# Autodesk Inventor assembly: plotter_new
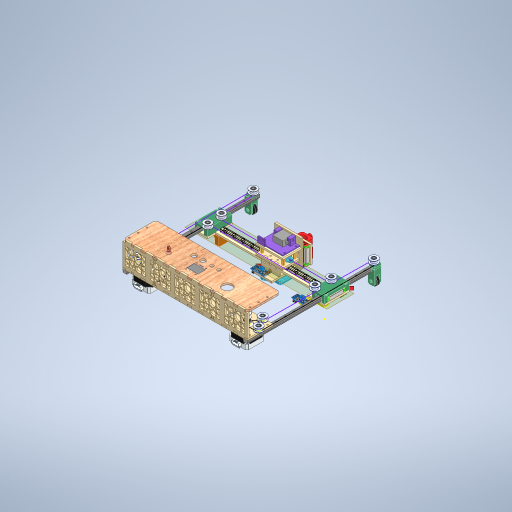
[picture p0: Inventor's stored thumbnail of the model, 512x512]
Saved by Autodesk Inventor 2024 (Build 280153000, 153)
## iProperties
Created: 2025-12-22
Part Number: plotter_new
Document SubType Name: Assembly
Designer: DELL
Author: DELL
## Documents named in this file (40)
- C:\Users\ejenie\reposGits\VSOSH25-26\models\plotter\plotter_actual\plotter_new.iam
- C:\Users\ejenie\reposGits\VSOSH25-26\models\plotter\plotter_actual\MGN9-H.ipt
- C:\Users\ejenie\reposGits\VSOSH25-26\models\plotter\plotter_actual\рельса.ipt
- C:\Users\ejenie\reposGits\VSOSH25-26\models\plotter\plotter_actual\Stepper motor Nema 17 (17HS2408).ipt
- C:\Users\ejenie\reposGits\VSOSH25-26\models\plotter\plotter_actual\центр_рейка.ipt
- C:\Users\ejenie\reposGits\VSOSH25-26\models\plotter\plotter_actual\креп_мотора.ipt
- C:\Users\ejenie\reposGits\VSOSH25-26\models\plotter\plotter_actual\Ролик с резьбой GT2 на моторы.ipt
- C:\Users\ejenie\reposGits\VSOSH25-26\models\plotter\plotter_actual\Сборка ролик с подшипником.ipt
- C:\Users\ejenie\reposGits\VSOSH25-26\models\plotter\plotter_actual\ограничитель.ipt
- C:\Users\ejenie\reposGits\VSOSH25-26\models\plotter\plotter_actual\рельса_центр.ipt
- C:\Users\ejenie\reposGits\VSOSH25-26\models\plotter\plotter_actual\Ролик с резьбой GT2 на моторы_MIR1.ipt
- C:\Users\ejenie\reposGits\VSOSH25-26\models\plotter\plotter_actual\Сборка ролик с подшипником_MIR3.ipt
- C:\Users\ejenie\reposGits\VSOSH25-26\models\plotter\plotter_actual\ограничитель_MIR.ipt
- C:\Users\ejenie\reposGits\VSOSH25-26\models\plotter\plotter_actual\креп_центр_м2.ipt
- C:\Users\ejenie\reposGits\VSOSH25-26\models\plotter\plotter_actual\Сборка ролик с подшипником_MIR4.ipt
- C:\Users\ejenie\reposGits\VSOSH25-26\models\plotter\plotter_actual\колесо.ipt
- C:\Users\ejenie\reposGits\VSOSH25-26\models\plotter\plotter_actual\концевик.ipt
- C:\Users\ejenie\reposGits\VSOSH25-26\models\plotter\plotter_actual\TCRT5000.ipt
- C:\Users\ejenie\reposGits\VSOSH25-26\models\plotter\plotter_actual\креп_опт.ipt
- C:\Users\ejenie\reposGits\VSOSH25-26\models\plotter\plotter_actual\креп_концевика.ipt
- C:\Users\ejenie\reposGits\VSOSH25-26\models\plotter\plotter_actual\креп_центр_м2_MIR1.ipt
- C:\Users\ejenie\reposGits\VSOSH25-26\models\plotter\plotter_actual\ремень.ipt
- C:\Users\ejenie\reposGits\VSOSH25-26\models\plotter\пол_каретки.ipt
- C:\Users\ejenie\reposGits\VSOSH25-26\models\plotter\стена_каретки.ipt
- C:\Users\ejenie\reposGits\VSOSH25-26\models\plotter\дно_каретки.ipt
- C:\Users\ejenie\reposGits\VSOSH25-26\models\plotter\plotter_actual\крепление_ремня_новое.ipt
- C:\Users\ejenie\reposGits\VSOSH25-26\models\plotter\plotter_actual\стойка.ipt
- C:\Users\ejenie\reposGits\VSOSH25-26\models\plotter\plotter_actual\креп_сервы.ipt
- C:\Users\ejenie\reposGits\VSOSH25-26\models\plotter\plotter_actual\JX Servo PDI-HV2006MG.ipt
- C:\Users\ejenie\reposGits\VSOSH25-26\models\plotter\plotter_actual\стена_для_рельс.ipt
- C:\Users\ejenie\reposGits\VSOSH25-26\models\plotter\plotter_actual\рельса_мини.ipt
- C:\Users\ejenie\reposGits\VSOSH25-26\models\plotter\plotter_actual\стена_движения_каретки_з.ipt
- C:\Users\ejenie\reposGits\VSOSH25-26\models\plotter\plotter_actual\креп_мотора (1).ipt
- C:\Users\ejenie\reposGits\VSOSH25-26\models\plotter\plotter_actual\креп_маркера.ipt
- C:\Users\ejenie\reposGits\VSOSH25-26\models\plotter\plotter_actual\каретки_потолок.ipt
- C:\Users\ejenie\reposGits\VSOSH25-26\models\plotter\plotter_actual\ширма.ipt
- C:\Users\ejenie\reposGits\VSOSH25-26\models\plotter\plotter_actual\line_sens_fixator.ipt
- C:\Users\ejenie\reposGits\VSOSH25-26\models\plotter\plotter_actual\I2C OLED 128Ч64 Display Module.ipt
- C:\Users\ejenie\reposGits\VSOSH25-26\models\plotter\plotter_actual\RCL371-1-1-12.ipt
- C:\Users\ejenie\reposGits\VSOSH25-26\models\plotter\plotter_actual\upor_koncevik.ipt
## Components (61 placed, 39 different names)
1. рельса:1 — Совмещение:1, Совмещение:11, Заподлицо:7, Совмещение:12, Заподлицо:9, Совмещение:62, Совмещение:63, Совмещение:90, Совмещение:91, Заподлицо:25, Совмещение:106
2. Stepper motor Nema 17 (17HS2408):2 — Заподлицо:7, Совмещение:12, Заподлицо:18, Совмещение:18, Заподлицо:25
3. рельса:2 — Заподлицо:13, Заподлицо:15, Совмещение:15, Совмещение:16, Заподлицо:16, Совмещение:50, Совмещение:51, Заподлицо:26, Совмещение:107
4. MGN9-H:2 — Совмещение:49
5. Stepper motor Nema 17 (17HS2408):3 — Заподлицо:15, Совмещение:15, Совмещение:60, Заподлицо:26, Совмещение:199
6. креп_мотора:1 — Заподлицо:18, Совмещение:19, Совмещение:96, Совмещение:97, Совмещение:98, Совмещение:99, Совмещение:244, Заподлицо:45, Заподлицо:46, Совмещение:299, Совмещение:300, Совмещение:301, Совмещение:302, Совмещение:303, Совмещение:304, Совмещение:305
7. Ролик с резьбой GT2 на моторы:1 — Совмещение:18, Совмещение:19
8. Сборка ролик с подшипником:1 — Совмещение:299, Совмещение:300
9. ограничитель:1 — Совмещение:90, Совмещение:91, Совмещение:92, Совмещение:93, Совмещение:102, Совмещение:103, Совмещение:106
10. Сборка ролик с подшипником:2 — Совмещение:92, Совмещение:93
11. Сборка ролик с подшипником:4 — Совмещение:160, Совмещение:161
12. Сборка ролик с подшипником:5 — Совмещение:162, Совмещение:166
13. рельса_центр:1 — Совмещение:37, Совмещение:38, Совмещение:52, Заподлицо:23, Совмещение:154
14. MGN9-H:3 — Совмещение:37, Совмещение:38, Совмещение:245, Совмещение:246, Совмещение:247
15. Ролик с резьбой GT2 на моторы_MIR1:1 — Совмещение:60, Совмещение:199
16. ограничитель_MIR:1 — Совмещение:39, Совмещение:40, Совмещение:50, Совмещение:51, Совмещение:104, Совмещение:105, Совмещение:107
17. Сборка ролик с подшипником_MIR3:2 — Совмещение:39, Совмещение:40
18. центр_рейка:1 — Совмещение:49, Совмещение:52, Заподлицо:23, Совмещение:66, Совмещение:67, Совмещение:127, Совмещение:136, Совмещение:146, Совмещение:147, Совмещение:149, Совмещение:155, Совмещение:156, Совмещение:157, Совмещение:158, Совмещение:200, Совмещение:201, Совмещение:202, Совмещение:322, Совмещение:323
19. MGN9-H:4 — Совмещение:62, Совмещение:63, Совмещение:66, Совмещение:67, Совмещение:127
20. Сборка ролик с подшипником_MIR4:1 — Совмещение:150, Совмещение:153
21. Сборка ролик с подшипником_MIR4:2 — Совмещение:152, Совмещение:165
22. Сборка ролик с подшипником:6 — Совмещение:96, Совмещение:97
23. Сборка ролик с подшипником:7 — Совмещение:98, Совмещение:99
24. Сборка ролик с подшипником:8 — Совмещение:301, Совмещение:302
25. колесо:1 — Совмещение:102, Совмещение:103
26. колесо:2 — Совмещение:104, Совмещение:105
27. концевик:1 — Совмещение:133, Совмещение:134, Совмещение:135
28. креп_центр_м2:1 — Совмещение:147, Совмещение:149, Совмещение:150, Совмещение:152, Совмещение:153, Совмещение:154, Совмещение:165
29. креп_концевика:2 — Совмещение:133, Совмещение:134, Совмещение:135, Совмещение:136, Совмещение:146, Совмещение:155
30. креп_центр_м2_MIR1:1 — Совмещение:156, Совмещение:157, Совмещение:158, Совмещение:160, Совмещение:161, Совмещение:162, Совмещение:166, Заподлицо:27
31. ремень:1 — Заподлицо:27
32. TCRT5000:3 — Совмещение:203, Заподлицо:31, Совмещение:204
33. креп_опт:1 — Совмещение:200, Совмещение:201, Совмещение:202, Совмещение:203, Заподлицо:31, Совмещение:204
34. креп_мотора (1):1 — Совмещение:244, Заподлицо:45, Заподлицо:46, Заподлицо:54, Совмещение:319, Совмещение:320, Совмещение:321
35. дно_каретки:1 — Совмещение:262, Совмещение:263, Заподлицо:50, Совмещение:264, Совмещение:265, Совмещение:270, Совмещение:271, Совмещение:272, Совмещение:310, Совмещение:311, Совмещение:312
36. пол_каретки:1 — Совмещение:245, Совмещение:246, Совмещение:247, Совмещение:248, Совмещение:250, Заподлицо:48, Совмещение:251, Заподлицо:49, Совмещение:252, Совмещение:253, Совмещение:254, Совмещение:255, Совмещение:256, Совмещение:257, Совмещение:258, Совмещение:259, Совмещение:260, Совмещение:268, Совмещение:269
37. стена_каретки:1 — Совмещение:248, Заподлицо:49, Совмещение:252
38. стена_каретки:2 — Совмещение:250, Заподлицо:48, Совмещение:251, Совмещение:262, Совмещение:263, Заподлицо:50, Совмещение:278, Совмещение:280
39. JX Servo PDI-HV2006MG:1 — Совмещение:275, Совмещение:306, Совмещение:307, Совмещение:308
40. креп_концевика:3 — Совмещение:270, Совмещение:271, Совмещение:272, Совмещение:293, Совмещение:294
41. TCRT5000:4 — Совмещение:264, Совмещение:265
42. стойка:1 — Совмещение:253, Совмещение:254
43. стойка:2 — Совмещение:255, Совмещение:256, Совмещение:267
44. стойка:3 — Совмещение:257, Совмещение:258, Совмещение:273
45. стойка:4 — Совмещение:259, Совмещение:260, Совмещение:266
46. стена_для_рельс:2 — Совмещение:278, Совмещение:280, Совмещение:281, Совмещение:282, Совмещение:283, Совмещение:284, Совмещение:285, Совмещение:286, Совмещение:309
47. стена_движения_каретки_з:2 — Совмещение:313, Совмещение:314, Совмещение:315, Совмещение:316, Совмещение:317, Совмещение:318
48. крепление_ремня_новое:1 — Совмещение:268, Совмещение:269
49. креп_сервы:2 — Совмещение:274, Заподлицо:51, Заподлицо:52, Совмещение:275, Совмещение:306, Совмещение:307, Совмещение:308
50. креп_маркера:1 — Совмещение:316, Совмещение:317, Совмещение:318
51. концевик:2 — Совмещение:293, Совмещение:294
52. каретки_потолок:1 — Совмещение:266, Совмещение:267, Совмещение:273, Совмещение:274, Заподлицо:51, Заподлицо:52, Совмещение:309
53. рельса_мини:3 — Совмещение:281, Совмещение:282, Совмещение:283, Совмещение:289, Совмещение:290
54. рельса_мини:4 — Совмещение:284, Совмещение:285, Совмещение:286, Совмещение:287, Совмещение:288
55. MGN9-H:7 — Совмещение:289, Совмещение:290, Заподлицо:53, Совмещение:313, Совмещение:314, Совмещение:315
56. MGN9-H:8 — Совмещение:287, Совмещение:288, Заподлицо:53
57. ширма:1 — Совмещение:303, Совмещение:304, Совмещение:305
58. line_sens_fixator:1 — Совмещение:310, Совмещение:311, Совмещение:312
59. I2C OLED 128Ч64 Display Module:1 — Заподлицо:54, Совмещение:319
60. RCL371-1-1-12:1 — Совмещение:320, Совмещение:321
61. upor_koncevik:1 — Совмещение:322, Совмещение:323
## Relationships (152: Mate 132, Flush 20)
- Совмещение:1 [Mate] (131.4 mm): рельса:1
- Совмещение:11 [Mate]: рельса:1
- Заподлицо:7 [Flush]: рельса:1 ↔ Stepper motor Nema 17 (17HS2408):2
- Совмещение:12 [Mate]: рельса:1 ↔ Stepper motor Nema 17 (17HS2408):2
- Заподлицо:9 [Flush] (150 mm): рельса:1
- [Mate]: рельса:2 ↔ MGN9-H:2
- [Mate] (-0.2 mm): рельса:2 ↔ MGN9-H:2
- Заподлицо:13 [Flush] (-150 mm): рельса:2
- Заподлицо:15 [Flush]: рельса:2 ↔ Stepper motor Nema 17 (17HS2408):3
- Совмещение:15 [Mate]: рельса:2 ↔ Stepper motor Nema 17 (17HS2408):3
- Совмещение:16 [Mate]: рельса:2
- Заподлицо:16 [Flush] (131.4 mm): рельса:2
- Заподлицо:18 [Flush]: Stepper motor Nema 17 (17HS2408):2 ↔ креп_мотора:1
- Совмещение:18 [Mate]: Stepper motor Nema 17 (17HS2408):2 ↔ Ролик с резьбой GT2 на моторы:1
- Совмещение:19 [Mate] (5 mm): креп_мотора:1 ↔ Ролик с резьбой GT2 на моторы:1
- Совмещение:37 [Mate]: рельса_центр:1 ↔ MGN9-H:3
- Совмещение:38 [Mate] (0.2 mm): рельса_центр:1 ↔ MGN9-H:3
- Совмещение:39 [Mate]: ограничитель_MIR:1 ↔ Сборка ролик с подшипником_MIR3:2
- Совмещение:40 [Mate]: ограничитель_MIR:1 ↔ Сборка ролик с подшипником_MIR3:2
- Совмещение:49 [Mate]: MGN9-H:2 ↔ центр_рейка:1
- Совмещение:50 [Mate]: рельса:2 ↔ ограничитель_MIR:1
- Совмещение:51 [Mate]: рельса:2 ↔ ограничитель_MIR:1
- Совмещение:52 [Mate]: рельса_центр:1 ↔ центр_рейка:1
- Заподлицо:23 [Flush] (-23.5 mm): рельса_центр:1 ↔ центр_рейка:1
- Совмещение:60 [Mate]: Stepper motor Nema 17 (17HS2408):3 ↔ Ролик с резьбой GT2 на моторы_MIR1:1
- Совмещение:62 [Mate]: рельса:1 ↔ MGN9-H:4
- Совмещение:63 [Mate] (-0.2 mm): рельса:1 ↔ MGN9-H:4
- Совмещение:66 [Mate]: центр_рейка:1 ↔ MGN9-H:4
- Совмещение:67 [Mate]: центр_рейка:1 ↔ MGN9-H:4
- Совмещение:90 [Mate]: рельса:1 ↔ ограничитель:1
- Совмещение:91 [Mate]: рельса:1 ↔ ограничитель:1
- Совмещение:92 [Mate]: ограничитель:1 ↔ Сборка ролик с подшипником:2
- Совмещение:93 [Mate]: ограничитель:1 ↔ Сборка ролик с подшипником:2
- Заподлицо:25 [Flush] (8 mm): рельса:1 ↔ Stepper motor Nema 17 (17HS2408):2
- Заподлицо:26 [Flush] (-8 mm): рельса:2 ↔ Stepper motor Nema 17 (17HS2408):3
- Совмещение:96 [Mate]: креп_мотора:1 ↔ Сборка ролик с подшипником:6
- Совмещение:97 [Mate]: креп_мотора:1 ↔ Сборка ролик с подшипником:6
- Совмещение:98 [Mate]: креп_мотора:1 ↔ Сборка ролик с подшипником:7
- Совмещение:99 [Mate]: креп_мотора:1 ↔ Сборка ролик с подшипником:7
- Совмещение:102 [Mate]: ограничитель:1 ↔ колесо:1
- Совмещение:103 [Mate]: ограничитель:1 ↔ колесо:1
- Совмещение:104 [Mate]: ограничитель_MIR:1 ↔ колесо:2
- Совмещение:105 [Mate]: ограничитель_MIR:1 ↔ колесо:2
- Совмещение:106 [Mate] (0.2 mm): рельса:1 ↔ ограничитель:1
- Совмещение:107 [Mate] (0.2 mm): рельса:2 ↔ ограничитель_MIR:1
- Совмещение:127 [Mate]: центр_рейка:1 ↔ MGN9-H:4
- Совмещение:133 [Mate]: концевик:1 ↔ креп_концевика:2
- Совмещение:134 [Mate]: концевик:1 ↔ креп_концевика:2
- Совмещение:135 [Mate]: концевик:1 ↔ креп_концевика:2
- Совмещение:136 [Mate]: центр_рейка:1 ↔ креп_концевика:2
- Совмещение:146 [Mate]: центр_рейка:1 ↔ креп_концевика:2
- Совмещение:147 [Mate]: центр_рейка:1 ↔ креп_центр_м2:1
- Совмещение:149 [Mate]: центр_рейка:1 ↔ креп_центр_м2:1
- Совмещение:150 [Mate]: Сборка ролик с подшипником_MIR4:1 ↔ креп_центр_м2:1
- Совмещение:152 [Mate]: Сборка ролик с подшипником_MIR4:2 ↔ креп_центр_м2:1
- Совмещение:153 [Mate]: Сборка ролик с подшипником_MIR4:1 ↔ креп_центр_м2:1
- Совмещение:154 [Mate] (5 mm): рельса_центр:1 ↔ креп_центр_м2:1
- Совмещение:155 [Mate]: центр_рейка:1 ↔ креп_концевика:2
- Совмещение:156 [Mate]: центр_рейка:1 ↔ креп_центр_м2_MIR1:1
- Совмещение:157 [Mate]: центр_рейка:1 ↔ креп_центр_м2_MIR1:1
- Совмещение:158 [Mate]: центр_рейка:1 ↔ креп_центр_м2_MIR1:1
- Совмещение:160 [Mate]: Сборка ролик с подшипником:4 ↔ креп_центр_м2_MIR1:1
- Совмещение:161 [Mate]: Сборка ролик с подшипником:4 ↔ креп_центр_м2_MIR1:1
- Совмещение:162 [Mate]: Сборка ролик с подшипником:5 ↔ креп_центр_м2_MIR1:1
- Совмещение:165 [Mate]: Сборка ролик с подшипником_MIR4:2 ↔ креп_центр_м2:1
- Совмещение:166 [Mate]: Сборка ролик с подшипником:5 ↔ креп_центр_м2_MIR1:1
- Заподлицо:27 [Flush]: креп_центр_м2_MIR1:1 ↔ ремень:1
- Совмещение:199 [Mate] (4 mm): Stepper motor Nema 17 (17HS2408):3 ↔ Ролик с резьбой GT2 на моторы_MIR1:1
- Совмещение:200 [Mate]: центр_рейка:1 ↔ креп_опт:1
- Совмещение:201 [Mate]: центр_рейка:1 ↔ креп_опт:1
- Совмещение:202 [Mate]: центр_рейка:1 ↔ креп_опт:1
- Совмещение:203 [Mate]: TCRT5000:3 ↔ креп_опт:1
- Заподлицо:31 [Flush]: TCRT5000:3 ↔ креп_опт:1
- Совмещение:204 [Mate]: TCRT5000:3 ↔ креп_опт:1
- Совмещение:244 [Mate] (50 mm): креп_мотора:1 ↔ креп_мотора (1):1
- Заподлицо:45 [Flush]: креп_мотора:1 ↔ креп_мотора (1):1
- Заподлицо:46 [Flush]: креп_мотора:1 ↔ креп_мотора (1):1
- Совмещение:245 [Mate]: MGN9-H:3 ↔ пол_каретки:1
- Совмещение:246 [Mate]: MGN9-H:3 ↔ пол_каретки:1
- Совмещение:247 [Mate]: MGN9-H:3 ↔ пол_каретки:1
- Совмещение:248 [Mate]: пол_каретки:1 ↔ стена_каретки:1
- Совмещение:250 [Mate]: пол_каретки:1 ↔ стена_каретки:2
- Заподлицо:48 [Flush]: пол_каретки:1 ↔ стена_каретки:2
- Совмещение:251 [Mate]: пол_каретки:1 ↔ стена_каретки:2
- Заподлицо:49 [Flush]: пол_каретки:1 ↔ стена_каретки:1
- Совмещение:252 [Mate]: пол_каретки:1 ↔ стена_каретки:1
- Совмещение:253 [Mate]: пол_каретки:1 ↔ стойка:1
- Совмещение:254 [Mate]: пол_каретки:1 ↔ стойка:1
- Совмещение:255 [Mate]: пол_каретки:1 ↔ стойка:2
- Совмещение:256 [Mate]: пол_каретки:1 ↔ стойка:2
- Совмещение:257 [Mate]: пол_каретки:1 ↔ стойка:3
- Совмещение:258 [Mate]: пол_каретки:1 ↔ стойка:3
- Совмещение:259 [Mate]: пол_каретки:1 ↔ стойка:4
- Совмещение:260 [Mate]: пол_каретки:1 ↔ стойка:4
- Совмещение:262 [Mate]: дно_каретки:1 ↔ стена_каретки:2
- Совмещение:263 [Mate]: дно_каретки:1 ↔ стена_каретки:2
- Заподлицо:50 [Flush]: дно_каретки:1 ↔ стена_каретки:2
- Совмещение:264 [Mate]: дно_каретки:1 ↔ TCRT5000:4
- Совмещение:265 [Mate]: дно_каретки:1 ↔ TCRT5000:4
- Совмещение:266 [Mate]: стойка:4 ↔ каретки_потолок:1
- Совмещение:267 [Mate]: стойка:2 ↔ каретки_потолок:1
- Совмещение:268 [Mate]: пол_каретки:1 ↔ крепление_ремня_новое:1
- Совмещение:269 [Mate]: пол_каретки:1 ↔ крепление_ремня_новое:1
- Совмещение:270 [Mate]: дно_каретки:1 ↔ креп_концевика:3
- Совмещение:271 [Mate]: дно_каретки:1 ↔ креп_концевика:3
- Совмещение:272 [Mate]: дно_каретки:1 ↔ креп_концевика:3
- Совмещение:273 [Mate]: стойка:3 ↔ каретки_потолок:1
- Совмещение:274 [Mate]: креп_сервы:2 ↔ каретки_потолок:1
- Заподлицо:51 [Flush] (2 mm): креп_сервы:2 ↔ каретки_потолок:1
- Заподлицо:52 [Flush]: креп_сервы:2 ↔ каретки_потолок:1
- Совмещение:275 [Mate]: JX Servo PDI-HV2006MG:1 ↔ креп_сервы:2
- Совмещение:278 [Mate]: стена_каретки:2 ↔ стена_для_рельс:2
- Совмещение:280 [Mate]: стена_каретки:2 ↔ стена_для_рельс:2
- Совмещение:281 [Mate]: стена_для_рельс:2 ↔ рельса_мини:3
- Совмещение:282 [Mate]: стена_для_рельс:2 ↔ рельса_мини:3
- Совмещение:283 [Mate]: стена_для_рельс:2 ↔ рельса_мини:3
- Совмещение:284 [Mate]: стена_для_рельс:2 ↔ рельса_мини:4
- Совмещение:285 [Mate]: стена_для_рельс:2 ↔ рельса_мини:4
- Совмещение:286 [Mate]: стена_для_рельс:2 ↔ рельса_мини:4
- Совмещение:287 [Mate]: рельса_мини:4 ↔ MGN9-H:8
- Совмещение:288 [Mate] (0.1 mm): рельса_мини:4 ↔ MGN9-H:8
- Совмещение:289 [Mate]: рельса_мини:3 ↔ MGN9-H:7
- Совмещение:290 [Mate] (0.1 mm): рельса_мини:3 ↔ MGN9-H:7
- Заподлицо:53 [Flush]: MGN9-H:7 ↔ MGN9-H:8
- Совмещение:293 [Mate]: креп_концевика:3 ↔ концевик:2
- Совмещение:294 [Mate]: креп_концевика:3 ↔ концевик:2
- Совмещение:299 [Mate]: креп_мотора:1 ↔ Сборка ролик с подшипником:1
- Совмещение:300 [Mate]: креп_мотора:1 ↔ Сборка ролик с подшипником:1
- Совмещение:301 [Mate]: креп_мотора:1 ↔ Сборка ролик с подшипником:8
- Совмещение:302 [Mate]: креп_мотора:1 ↔ Сборка ролик с подшипником:8
- Совмещение:303 [Mate]: креп_мотора:1 ↔ ширма:1
- Совмещение:304 [Mate]: креп_мотора:1 ↔ ширма:1
- Совмещение:305 [Mate]: креп_мотора:1 ↔ ширма:1
- Совмещение:306 [Mate]: JX Servo PDI-HV2006MG:1 ↔ креп_сервы:2
- Совмещение:307 [Mate]: JX Servo PDI-HV2006MG:1 ↔ креп_сервы:2
- Совмещение:308 [Mate]: JX Servo PDI-HV2006MG:1 ↔ креп_сервы:2
- Совмещение:309 [Mate]: стена_для_рельс:2 ↔ каретки_потолок:1
- Совмещение:310 [Mate]: дно_каретки:1 ↔ line_sens_fixator:1
- Совмещение:311 [Mate]: дно_каретки:1 ↔ line_sens_fixator:1
- Совмещение:312 [Mate]: дно_каретки:1 ↔ line_sens_fixator:1
- Совмещение:313 [Mate]: стена_движения_каретки_з:2 ↔ MGN9-H:7
- Совмещение:314 [Mate]: стена_движения_каретки_з:2 ↔ MGN9-H:7
- Совмещение:315 [Mate]: стена_движения_каретки_з:2 ↔ MGN9-H:7
- Совмещение:316 [Mate]: стена_движения_каретки_з:2 ↔ креп_маркера:1
- Совмещение:317 [Mate]: стена_движения_каретки_з:2 ↔ креп_маркера:1
- Совмещение:318 [Mate]: стена_движения_каретки_з:2 ↔ креп_маркера:1
- Заподлицо:54 [Flush]: креп_мотора (1):1 ↔ I2C OLED 128Ч64 Display Module:1
- Совмещение:319 [Mate]: креп_мотора (1):1 ↔ I2C OLED 128Ч64 Display Module:1
- Совмещение:320 [Mate]: креп_мотора (1):1 ↔ RCL371-1-1-12:1
- Совмещение:321 [Mate]: креп_мотора (1):1 ↔ RCL371-1-1-12:1
- Совмещение:322 [Mate]: центр_рейка:1 ↔ upor_koncevik:1
- Совмещение:323 [Mate]: центр_рейка:1 ↔ upor_koncevik:1
## Named parameters: d34_d9 = 0 mm, d35_d10 = -0.2 mm
